# Autodesk Inventor assembly: transmitter_case
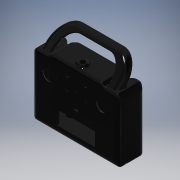
[picture p0: Inventor's stored thumbnail of the model, 180x180]
Saved by Autodesk Inventor 2019.4 (Build 234330000, 330)
## iProperties
Created: 2020-07-20
Part Number: transmitter_case
Document SubType Name: Assembly
Designer: alex_
Author: alex_
## Documents named in this file (4)
- G:\3D Modelling\3D Models\Spitfire Transmitter\transmitter_case.iam
- G:\3D Modelling\3D Models\Spitfire Transmitter\transmitter_case_bottom.ipt
- G:\3D Modelling\3D Models\Spitfire Transmitter\transmitter_case_top.ipt
- G:\3D Modelling\3D Models\Spitfire Transmitter\battery_cover.ipt
## Components (3 placed, 3 different names)
1. transmitter_case_bottom:1 — Rigid:2, Rigid:3
2. transmitter_case_top:1 — Rigid:3
3. battery_cover:1 — Rigid:2
## Relationships (2: WeldJoint 2)
- Rigid:2 [WeldJoint]: transmitter_case_bottom:1 ↔ battery_cover:1
- Rigid:3 [WeldJoint]: transmitter_case_bottom:1 ↔ transmitter_case_top:1
